# Autodesk Inventor assembly: Index_Finger_assembly_1
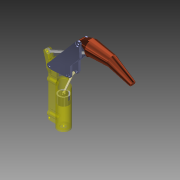
[picture p0: Inventor's stored thumbnail of the model, 180x180]
Saved by Autodesk Inventor 2015 (Build 190159000, 159)
## iProperties
Created: 2016-07-06
Part Number: Index_Finger_assembly_1
Document SubType Name: Assembly
Designer: Neelotpal Nag
Author: Neelotpal Nag
## Documents named in this file (7)
- D:\NEEL BACKUP\DISA 2016\Fingers 1\Index_Finger_assembly_1.iam
- D:\NEEL BACKUP\DISA 2016\Fingers 1\Finger_Lower_main_1.ipt
- D:\NEEL BACKUP\DISA 2016\Fingers 1\Restrain_Pin_1.ipt
- D:\NEEL BACKUP\DISA 2016\Fingers 1\Shaft_Piston.ipt
- D:\NEEL BACKUP\DISA 2016\Fingers 1\Index_Upper_main_1.ipt
- D:\NEEL BACKUP\DISA 2016\Fingers 1\Base_Cylinder_11mm.ipt
- D:\NEEL BACKUP\DISA 2016\Fingers 1\Cylinder_10.5mm.ipt
## Components (6 placed, 6 different names)
1. Finger_Lower_main_1:1 — Mate:15, Mate:18, Mate:19, Mate:25, Mate:27
2. Shaft_Piston:1 — Mate:15, Mate:22, Mate:23, Angle:1
3. Restrain_Pin_1:1 — Mate:20, Mate:24, Mate:26
4. Index_Upper_main_1:1 — Mate:18, Mate:19, Mate:20, Mate:24
5. Base_Cylinder_11mm:1 — Mate:21, Angle:1, Mate:25, Mate:26, Mate:27
6. Cylinder_10.5mm:1 — Mate:21, Mate:22, Mate:23
## Relationships (12: Mate 11, Angle 1)
- Mate:15: Finger_Lower_main_1:1 ↔ Shaft_Piston:1
- Mate:18: Finger_Lower_main_1:1 ↔ Index_Upper_main_1:1
- Mate:19 (0.5 mm): Finger_Lower_main_1:1 ↔ Index_Upper_main_1:1
- Mate:20: Restrain_Pin_1:1 ↔ Index_Upper_main_1:1
- Mate:21: Base_Cylinder_11mm:1 ↔ Cylinder_10.5mm:1
- Mate:22: Shaft_Piston:1 ↔ Cylinder_10.5mm:1
- Mate:23: Shaft_Piston:1 ↔ Cylinder_10.5mm:1
- Mate:24 (0.3 mm): Restrain_Pin_1:1 ↔ Index_Upper_main_1:1
- Angle:1 (0 deg): Shaft_Piston:1 ↔ Base_Cylinder_11mm:1
- Mate:25: Finger_Lower_main_1:1 ↔ Base_Cylinder_11mm:1
- Mate:26: Restrain_Pin_1:1 ↔ Base_Cylinder_11mm:1
- Mate:27: Finger_Lower_main_1:1 ↔ Base_Cylinder_11mm:1
